# Autodesk Inventor assembly: slides with motors
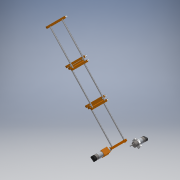
[picture p0: Inventor's stored thumbnail of the model, 180x180]
Saved by Autodesk Inventor 2019 (Build 230136000, 136)
## iProperties
Created: 2019-03-30
Part Number: slides with motors
Document SubType Name: Assembly
Designer: User
Author: User
## Documents named in this file (6)
- C:\Robotics\CAD\2019-20_CAD\Linear Slides\slides with motors.iam
- C:\Robotics\CAD\2019-20_CAD\Linear Slides\Linear slides.iam
- C:\Robotics\CAD\COTSParts\Motors\am-3643 NeveRest Sport, 104-1 with Motor.ipt
- C:\Robotics\CAD\COTSParts\Motors\am-3102NeveRest20 (1).ipt
- C:\Robotics\CAD\COTSParts\Tetrix\tetrix-motor-mounts-1.snapshot.1\Tetrex 2pc motor mount.ipt
- C:\Robotics\CAD\2016-17_CAD\LiftPully.ipt
## Components (9 placed, 5 different names)
1. Linear slides:1 [sub-assembly] — Mate:1, Mate:2, Mate:3, Mate:5, Mate:6, Mate:7, Mate:8, Mate:9, Mate:10, Mate:11, Mate:12, Mate:13, Mate:14
2. am-3643 NeveRest Sport, 104-1 with Motor:1 — Mate:1, Mate:2, Flush:1, Mate:4
3. am-3102NeveRest20 (1):1 — Insert:1, Mate:3
4. Tetrex 2pc motor mount:1 — Insert:1, Flush:1, Mate:4
5. LiftPully:1 — Mate:9, Mate:10
6. LiftPully:2 — Mate:5, Mate:6
7. LiftPully:3 — Mate:11, Mate:14
8. LiftPully:4 — Mate:12, Mate:13
9. LiftPully:5 — Mate:7, Mate:8
## Relationships (16: Mate 14, Insert 1, Flush 1)
- Mate:1: Linear slides:1 ↔ am-3643 NeveRest Sport, 104-1 with Motor:1
- Mate:2: Linear slides:1 ↔ am-3643 NeveRest Sport, 104-1 with Motor:1
- Insert:1: am-3102NeveRest20 (1):1 ↔ Tetrex 2pc motor mount:1
- Flush:1: am-3643 NeveRest Sport, 104-1 with Motor:1 ↔ Tetrex 2pc motor mount:1
- Mate:3: Linear slides:1 ↔ am-3102NeveRest20 (1):1
- Mate:4: am-3643 NeveRest Sport, 104-1 with Motor:1 ↔ Tetrex 2pc motor mount:1
- Mate:5: Linear slides:1 ↔ LiftPully:2
- Mate:6: Linear slides:1 ↔ LiftPully:2
- Mate:7: Linear slides:1 ↔ LiftPully:5
- Mate:8: Linear slides:1 ↔ LiftPully:5
- Mate:9: Linear slides:1 ↔ LiftPully:1
- Mate:10: Linear slides:1 ↔ LiftPully:1
- Mate:11: Linear slides:1 ↔ LiftPully:3
- Mate:12: Linear slides:1 ↔ LiftPully:4
- Mate:13: Linear slides:1 ↔ LiftPully:4
- Mate:14: Linear slides:1 ↔ LiftPully:3
